# Autodesk Inventor assembly: 付け根ロール_1
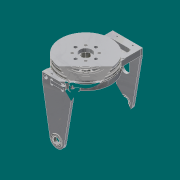
[picture p0: Inventor's stored thumbnail of the model, 180x180]
Saved by Autodesk Inventor 2016 (Build 200138000, 138)
## iProperties
Created: 2016-05-01
Part Number: 付け根ロール_1
Document SubType Name: Assembly
Designer: hiroaki
Mass: 95.2431 g
Surface Area: 199.324 cm^2
Volume: 15.6569 cm^3
Density: 6.08314 g/cm^3
Author: hiroaki
## Documents named in this file (10)
- C:\Users\hiro\Documents\kenkyuu\二足\二足ver6.0\下半身_160823\付け根ロール\付け根ロール_6.iam
- C:\Users\hiro\Documents\kenkyuu\二足\二足ver6.0\既製品\NSK_RB_MF85ZZ\MF85ZZ.iam
- C:\Users\hiro\Documents\kenkyuu\二足\二足ver6.0\既製品\BA2542\core_BA2542.ipt
- C:\Users\hiro\Documents\kenkyuu\二足\二足ver6.0\既製品\BA2542\washer_BA2542.ipt
- C:\Users\hiro\Documents\kenkyuu\二足\二足ver6.0\既製品\SLCG5_5-6.ipt
- C:\Users\hiro\Documents\kenkyuu\二足\二足ver6.0\下半身_160823\付け根ロール\付け根ロール_サブフレーム_6_4.ipt
- C:\Users\hiro\Documents\kenkyuu\二足\二足ver6.0\下半身_160823\付け根ロール\付け根ロール_メインフレーム_6_1.ipt
- C:\Users\hiro\Documents\kenkyuu\二足\二足ver6.0\下半身_160823\付け根ロール\付け根ロール_サブフレーム_6_5.ipt
- C:\Users\hiro\Documents\kenkyuu\二足\二足ver6.0\下半身_160823\付け根ロール\付け根ロール_サブフレーム_6_6.ipt
- C:\Users\hiro\Documents\kenkyuu\二足\二足ver6.0\既製品\新規購入\D4050-9120B.ipt
## Components (14 placed, 9 different names)
1. MF85ZZ:1 [sub-assembly] — 挿入:56
2. core_BA2542:1 — 挿入:30
3. core_BA2542:2 — 挿入:51
4. washer_BA2542:1 — 挿入:30, 挿入:46
5. SLCG5_5-6:1 — 挿入:35, 挿入:48
6. SLCG5_5-6:2 — 挿入:45, 挿入:49
7. SLCG5_5-6:3 — 挿入:36, 挿入:47
8. SLCG5_5-6:4 — 挿入:37, 挿入:50
9. 付け根ロール_サブフレーム_6_4:1 — 挿入:35, 挿入:36, 挿入:37, 挿入:45, 挿入:51
10. 付け根ロール_メインフレーム_6_1:1 — 挿入:46, 挿入:47, 挿入:48, 挿入:49, 挿入:50, 挿入:52, 挿入:53, 挿入:54, 挿入:55
11. 付け根ロール_サブフレーム_6_5:1 — 挿入:52, 挿入:53, 挿入:57
12. 付け根ロール_サブフレーム_6_6:1 — 挿入:54, 挿入:55, 挿入:56
13. D4050-9120B:1 — 挿入:58
14. MF85ZZ:2 [sub-assembly] — 挿入:57, 挿入:58
## Relationships (18: Insert 18)
- 挿入:30 [Insert]: core_BA2542:1 ↔ washer_BA2542:1
- 挿入:35 [Insert]: SLCG5_5-6:1 ↔ 付け根ロール_サブフレーム_6_4:1
- 挿入:36 [Insert]: SLCG5_5-6:3 ↔ 付け根ロール_サブフレーム_6_4:1
- 挿入:37 [Insert]: SLCG5_5-6:4 ↔ 付け根ロール_サブフレーム_6_4:1
- 挿入:45 [Insert]: SLCG5_5-6:2 ↔ 付け根ロール_サブフレーム_6_4:1
- 挿入:46 [Insert]: washer_BA2542:1 ↔ 付け根ロール_メインフレーム_6_1:1
- 挿入:47 [Insert]: SLCG5_5-6:3 ↔ 付け根ロール_メインフレーム_6_1:1
- 挿入:48 [Insert]: SLCG5_5-6:1 ↔ 付け根ロール_メインフレーム_6_1:1
- 挿入:49 [Insert]: SLCG5_5-6:2 ↔ 付け根ロール_メインフレーム_6_1:1
- 挿入:50 [Insert]: SLCG5_5-6:4 ↔ 付け根ロール_メインフレーム_6_1:1
- 挿入:51 [Insert]: core_BA2542:2 ↔ 付け根ロール_サブフレーム_6_4:1
- 挿入:52 [Insert]: 付け根ロール_メインフレーム_6_1:1 ↔ 付け根ロール_サブフレーム_6_5:1
- 挿入:53 [Insert]: 付け根ロール_メインフレーム_6_1:1 ↔ 付け根ロール_サブフレーム_6_5:1
- 挿入:54 [Insert]: 付け根ロール_メインフレーム_6_1:1 ↔ 付け根ロール_サブフレーム_6_6:1
- 挿入:55 [Insert]: 付け根ロール_メインフレーム_6_1:1 ↔ 付け根ロール_サブフレーム_6_6:1
- 挿入:56 [Insert]: MF85ZZ:1 ↔ 付け根ロール_サブフレーム_6_6:1
- 挿入:57 [Insert]: 付け根ロール_サブフレーム_6_5:1 ↔ MF85ZZ:2
- 挿入:58 [Insert]: D4050-9120B:1 ↔ MF85ZZ:2
